# Autodesk Inventor assembly: Project Assembly
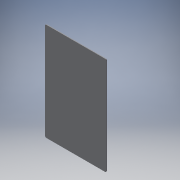
[picture p0: Inventor's stored thumbnail of the model, 180x180]
Saved by Autodesk Inventor 2019 (Build 230136000, 136)
## iProperties
Created: 2021-06-06
Part Number: Project Assembly
Document SubType Name: Assembly
Designer: micha
Author: micha
## Documents named in this file (17)
- D:\Files\ASU - Faculty of Engineering\Semester 10 - Spring 2021\Industrial Mechanisms and Robotics - MCT331\Four Bar Gripper Project\Project Assembly.iam
- D:\Files\ASU - Faculty of Engineering\Semester 10 - Spring 2021\Industrial Mechanisms and Robotics - MCT331\Four Bar Gripper Project\Base.ipt
- D:\Files\ASU - Faculty of Engineering\Semester 10 - Spring 2021\Industrial Mechanisms and Robotics - MCT331\Four Bar Gripper Project\NEMA 23 - 56mm.iam
- D:\Files\ASU - Faculty of Engineering\Semester 10 - Spring 2021\Industrial Mechanisms and Robotics - MCT331\Four Bar Gripper Project\nema23-mounting-L-bracket.ipt
- D:\Files\ASU - Faculty of Engineering\Semester 10 - Spring 2021\Industrial Mechanisms and Robotics - MCT331\Four Bar Gripper Project\Project Assembly\Design Accelerator\Spur Gears2.iam
- D:\Files\ASU - Faculty of Engineering\Semester 10 - Spring 2021\Industrial Mechanisms and Robotics - MCT331\Four Bar Gripper Project\Ruland_PCMR25-10-6-A.ipt
- D:\Files\ASU - Faculty of Engineering\Semester 10 - Spring 2021\Industrial Mechanisms and Robotics - MCT331\Four Bar Gripper Project\Small Gear Shaft.ipt
- D:\Files\ASU - Faculty of Engineering\Semester 10 - Spring 2021\Industrial Mechanisms and Robotics - MCT331\Four Bar Gripper Project\KP08\KP08_BearingV.iam
- D:\Files\ASU - Faculty of Engineering\Semester 7 - Fall 2019\MCT381 - Design of Mechatronic Systems (1)\Production Line Project\MCT381_Disassembly_26Nov\Workspaces\Workspace\Bearing Seat 8mm.ipt
- D:\Files\ASU - Faculty of Engineering\Semester 10 - Spring 2021\Industrial Mechanisms and Robotics - MCT331\Four Bar Gripper Project\Large Gear Shaft.ipt
- D:\Files\ASU - Faculty of Engineering\Semester 10 - Spring 2021\Industrial Mechanisms and Robotics - MCT331\Four Bar Gripper Project\Bearing 10mm.ipt
- D:\Files\ASU - Faculty of Engineering\Semester 10 - Spring 2021\Industrial Mechanisms and Robotics - MCT331\Four Bar Gripper Project\Bearing Seats 10mm.ipt
- D:\Files\ASU - Faculty of Engineering\Semester 10 - Spring 2021\Industrial Mechanisms and Robotics - MCT331\Four Bar Gripper Project\ScaledAssembly.ipt
- D:\Files\ASU - Faculty of Engineering\Semester 10 - Spring 2021\Industrial Mechanisms and Robotics - MCT331\Four Bar Gripper Project\Fourbar-Crank.ipt
- D:\Files\ASU - Faculty of Engineering\Semester 10 - Spring 2021\Industrial Mechanisms and Robotics - MCT331\Four Bar Gripper Project\Fourbar-Coupler.ipt
- D:\Files\ASU - Faculty of Engineering\Semester 10 - Spring 2021\Industrial Mechanisms and Robotics - MCT331\Four Bar Gripper Project\Fourbar-Rocker.ipt
- D:\Files\ASU - Faculty of Engineering\Semester 10 - Spring 2021\Industrial Mechanisms and Robotics - MCT331\Four Bar Gripper Project\Rocker Base Joint.ipt
## Components (19 placed, 16 different names)
1. Base:1 — Mate:2, Angle:2, Flush:1, Angle:3, Mate:13, Flush:2, Angle:4, Mate:21, Mate:26, Mate:36, Mate:39, Mate:42
2. NEMA 23 - 56mm:1 [sub-assembly] — Mate:1, Mate:3, Angle:1, Mate:4, Mate:5, Mate:6
3. nema23-mounting-L-bracket:1 — Mate:1, Mate:2, Mate:3, Angle:1, Angle:2, Flush:1, Flush:2
4. Spur Gears:1 [sub-assembly] — Mate:4, Mate:9, Mate:10, Flush:3, Mate:16, Mate:28
5. Ruland_PCMR25-10-6-A:1 — Mate:5, Mate:6, Mate:8
6. Small Gear Shaft:1 — Mate:8, Mate:9, Mate:10, Mate:11, Mate:12
7. KP08_BearingV:1 [sub-assembly] — Mate:11, Mate:12, Angle:3, Mate:14, Mate:15
8. Bearing Seat 8mm:1 — Mate:13, Mate:14, Mate:15
9. Large Gear Shaft:1 — Flush:3, Mate:16, Mate:17, Mate:18, Mate:19, Mate:20, Mate:29
10. Bearing 10mm:1 — Mate:17, Mate:18, Angle:4, Flush:4, Mate:22, Mate:23, Mate:24
11. Bearing 10mm:2 — Mate:19, Mate:20, Flush:4, Mate:25, Mate:27
12. Bearing Seats 10mm:1 — Mate:21, Mate:22, Mate:23, Mate:24
13. Bearing Seats 10mm:2 — Mate:25, Mate:26, Mate:27
14. ScaledAssembly:1 — Mate:34, Mate:35, Flush:5
15. Fourbar-Crank:1 — Mate:28, Mate:29, Mate:30, Mate:31
16. Fourbar-Coupler:1 — Mate:30, Mate:31, Mate:32, Mate:33
17. Fourbar-Rocker:1 — Mate:32, Mate:33, Mate:34, Mate:35, Flush:5, Mate:37, Mate:38, Mate:40, Mate:41
18. Rocker Base Joint:1 — Mate:36, Mate:37, Mate:38
19. Rocker Base Joint:2 — Mate:39, Mate:40, Mate:41, Mate:42
## Relationships (50: Mate 41, Flush 5, Angle 4)
- Mate:1: NEMA 23 - 56mm:1 ↔ nema23-mounting-L-bracket:1
- Mate:2: Base:1 ↔ nema23-mounting-L-bracket:1
- Mate:3: NEMA 23 - 56mm:1 ↔ nema23-mounting-L-bracket:1
- Angle:1 (0 deg): NEMA 23 - 56mm:1 ↔ nema23-mounting-L-bracket:1
- Angle:2 (0 deg): Base:1 ↔ nema23-mounting-L-bracket:1
- Mate:4: NEMA 23 - 56mm:1 ↔ Spur Gears:1
- Flush:1 (75 mm): Base:1 ↔ nema23-mounting-L-bracket:1
- Mate:5: NEMA 23 - 56mm:1 ↔ Ruland_PCMR25-10-6-A:1
- Mate:6 (-7 mm): NEMA 23 - 56mm:1 ↔ Ruland_PCMR25-10-6-A:1
- Mate:8: Ruland_PCMR25-10-6-A:1 ↔ Small Gear Shaft:1
- Mate:9: Spur Gears:1 ↔ Small Gear Shaft:1
- Mate:10: Spur Gears:1 ↔ Small Gear Shaft:1
- Mate:11: Small Gear Shaft:1 ↔ KP08_BearingV:1
- Mate:12: Small Gear Shaft:1 ↔ KP08_BearingV:1
- Angle:3 (180 deg): Base:1 ↔ KP08_BearingV:1
- Mate:13: Base:1 ↔ Bearing Seat 8mm:1
- Mate:14: KP08_BearingV:1 ↔ Bearing Seat 8mm:1
- Mate:15: KP08_BearingV:1 ↔ Bearing Seat 8mm:1
- Flush:2 (80 mm): Base:1 ↔ nema23-mounting-L-bracket:1
- Flush:3: Spur Gears:1 ↔ Large Gear Shaft:1
- Mate:16: Spur Gears:1 ↔ Large Gear Shaft:1
- Mate:17: Large Gear Shaft:1 ↔ Bearing 10mm:1
- Mate:18: Large Gear Shaft:1 ↔ Bearing 10mm:1
- Angle:4 (180 deg): Base:1 ↔ Bearing 10mm:1
- Mate:19: Large Gear Shaft:1 ↔ Bearing 10mm:2
- Mate:20: Large Gear Shaft:1 ↔ Bearing 10mm:2
- Flush:4: Bearing 10mm:1 ↔ Bearing 10mm:2
- Mate:21: Base:1 ↔ Bearing Seats 10mm:1
- Mate:22: Bearing 10mm:1 ↔ Bearing Seats 10mm:1
- Mate:23: Bearing 10mm:1 ↔ Bearing Seats 10mm:1
- Mate:24: Bearing 10mm:1 ↔ Bearing Seats 10mm:1
- Mate:25: Bearing 10mm:2 ↔ Bearing Seats 10mm:2
- Mate:26: Base:1 ↔ Bearing Seats 10mm:2
- Mate:27: Bearing 10mm:2 ↔ Bearing Seats 10mm:2
- Mate:28: Spur Gears:1 ↔ Fourbar-Crank:1
- Mate:29: Large Gear Shaft:1 ↔ Fourbar-Crank:1
- Mate:30: Fourbar-Crank:1 ↔ Fourbar-Coupler:1
- Mate:31: Fourbar-Crank:1 ↔ Fourbar-Coupler:1
- Mate:32: Fourbar-Coupler:1 ↔ Fourbar-Rocker:1
- Mate:33: Fourbar-Coupler:1 ↔ Fourbar-Rocker:1
- Mate:34: ScaledAssembly:1 ↔ Fourbar-Rocker:1
- Mate:35 (-100 mm): ScaledAssembly:1 ↔ Fourbar-Rocker:1
- Flush:5: ScaledAssembly:1 ↔ Fourbar-Rocker:1
- Mate:36: Base:1 ↔ Rocker Base Joint:1
- Mate:37: Fourbar-Rocker:1 ↔ Rocker Base Joint:1
- Mate:38: Fourbar-Rocker:1 ↔ Rocker Base Joint:1
- Mate:39: Base:1 ↔ Rocker Base Joint:2
- Mate:40: Fourbar-Rocker:1 ↔ Rocker Base Joint:2
- Mate:41: Fourbar-Rocker:1 ↔ Rocker Base Joint:2
- Mate:42 (-475 mm): Base:1 ↔ Rocker Base Joint:2
